# Autodesk Inventor assembly: teljes3
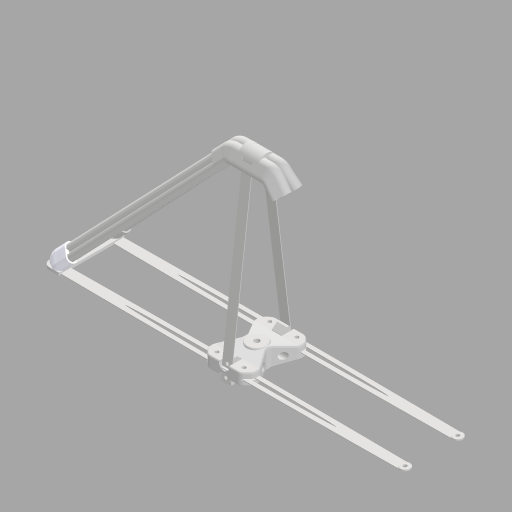
[picture p0: Inventor's stored thumbnail of the model, 512x512]
Saved by Autodesk Inventor 2023 (Build 270158000, 158)
## iProperties
Created: 2022-11-11
Part Number: teljes3
Document SubType Name: Assembly
Designer: gd1
Author: gd1
## Documents named in this file (7)
- C:\Users\gd1\3D Objects\3D nagyteherbírású híd\Híd\H-d\teljes8.iam
- C:\Users\gd1\3D Objects\3D nagyteherbírású híd\Híd\H-d\45 fok középre_talp másolata.ipt
- C:\Users\gd1\3D Objects\3D nagyteherbírású híd\Híd\H-d\palca 325mm.ipt
- C:\Users\gd1\3D Objects\3D nagyteherbírású híd\Híd\H-d\kozepcsati2.iam
- C:\Users\gd1\3D Objects\3D nagyteherbírású híd\Híd\H-d\szalag5.ipt
- C:\Users\gd1\3D Objects\3D nagyteherbírású híd\Híd\H-d\kozepso_csomopont2.0.ipt
- C:\Users\gd1\3D Objects\3D nagyteherbírású híd\Híd\H-d\szalag3.ipt
## Components (8 placed, 6 different names)
1. 45 fok középre_talp másolata:1 — Rotational:1, Rotational:2, Rigid:1, Rotational:4
2. palca 325mm:1 — Rotational:1
3. palca 325mm:2 — Rotational:2, Mate:1
4. kozepcsati2:1 [sub-assembly] — Mate:1, Mate:2
5. szalag5:1 — Mate:2, Rotational:3
6. kozepso_csomopont2.0:1 — Rotational:3
7. szalag3:1 — Rigid:1
8. szalag3:2 — Rotational:4
## Relationships (7: RevoluteJoint 4, Mate 2, WeldJoint 1)
- Rotational:1 [RevoluteJoint]: 45 fok középre_talp másolata:1 ↔ palca 325mm:1
- Rotational:2 [RevoluteJoint]: 45 fok középre_talp másolata:1 ↔ palca 325mm:2
- Mate:1: palca 325mm:2 ↔ kozepcsati2:1
- Mate:2: kozepcsati2:1 ↔ szalag5:1
- Rotational:3 [RevoluteJoint]: szalag5:1 ↔ kozepso_csomopont2.0:1
- Rigid:1 [WeldJoint]: 45 fok középre_talp másolata:1 ↔ szalag3:1
- Rotational:4 [RevoluteJoint]: 45 fok középre_talp másolata:1 ↔ szalag3:2
